# Autodesk Inventor assembly: jorge's assembly
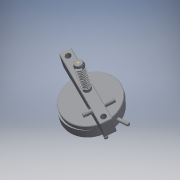
[picture p0: Inventor's stored thumbnail of the model, 180x180]
Saved by Autodesk Inventor 2017 (Build 210142000, 142)
## iProperties
Created: 2017-04-26
Part Number: jorge's assembly
Document SubType Name: Assembly
Designer: 167942
Author: 167942
## Documents named in this file (10)
- C:\Users\167942.FCBOE\Desktop\jorge's assembly.iam
- C:\Users\167942.FCBOE\Desktop\Part3.ipt
- C:\Users\167942.FCBOE\Desktop\Part4.ipt
- C:\Users\167942.FCBOE\Desktop\handle pivot pin.ipt
- C:\Users\167942.FCBOE\Downloads\upper die center support.ipt
- C:\Users\167942.FCBOE\Downloads\upper die pressure ring.ipt
- C:\Users\167942.FCBOE\Downloads\upper die center pin.ipt
- C:\Users\167942.FCBOE\Desktop\snap ring.ipt
- C:\Users\167942.FCBOE\Desktop\spring.ipt
- C:\Users\167942.FCBOE\Desktop\screw.ipt
## Components (9 placed, 9 different names)
1. Part3:1 — Rotational:4
2. Part4:1 — Rotational:5, Rotational:6
3. handle pivot pin:1 — Cylindrical:1
4. upper die center support:1 — Cylindrical:1, Rigid:1, Rotational:3
5. upper die pressure ring:1 — Rotational:3, Rotational:4, Rotational:5
6. upper die center pin:1 — Rotational:1, Rotational:2, Rigid:1
7. snap ring:1 — Rotational:1
8. spring:1 — Rotational:2
9. screw:1 — Rotational:6
## Relationships (8: RevoluteJoint 6, CylindricalJoint 1, WeldJoint 1)
- Rotational:1 [RevoluteJoint]: upper die center pin:1 ↔ snap ring:1
- Rotational:2 [RevoluteJoint]: upper die center pin:1 ↔ spring:1
- Cylindrical:1: handle pivot pin:1 ↔ upper die center support:1
- Rigid:1 [WeldJoint]: upper die center support:1 ↔ upper die center pin:1
- Rotational:3 [RevoluteJoint]: upper die center support:1 ↔ upper die pressure ring:1
- Rotational:4 [RevoluteJoint]: Part3:1 ↔ upper die pressure ring:1
- Rotational:5 [RevoluteJoint]: Part4:1 ↔ upper die pressure ring:1
- Rotational:6 [RevoluteJoint]: Part4:1 ↔ screw:1
